# Autodesk Inventor assembly: noseAssembly
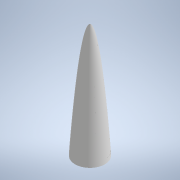
[picture p0: Inventor's stored thumbnail of the model, 180x180]
Saved by Autodesk Inventor 2020.3 (Build 243373000, 373)
## iProperties
Created: 2021-03-12
Part Number: noseAssembly
Document SubType Name: Assembly
Designer: 0x6f736f646f
Author: 0x6f736f646f
## Documents named in this file (3)
- C:\Users\0x6f736f646f\OneDrive\Documents\Inventor\Nakuja project\noseAssembly.iam
- C:\Users\0x6f736f646f\OneDrive\Documents\Inventor\Nakuja project\nose-basepart1.ipt
- C:\Users\0x6f736f646f\OneDrive\Documents\Inventor\Nakuja project\nose-toppart1.ipt
## Components (2 placed, 2 different names)
1. nose-basepart1:1 — Mate:1, Mate:2, Mate:3, Mate:4
2. nose-toppart1:1 — Mate:1, Mate:2, Mate:3, Mate:4
## Relationships (4: Mate 4)
- Mate:1: nose-basepart1:1 ↔ nose-toppart1:1
- Mate:2: nose-basepart1:1 ↔ nose-toppart1:1
- Mate:3: nose-basepart1:1 ↔ nose-toppart1:1
- Mate:4: nose-basepart1:1 ↔ nose-toppart1:1
